# Autodesk Inventor assembly: outer
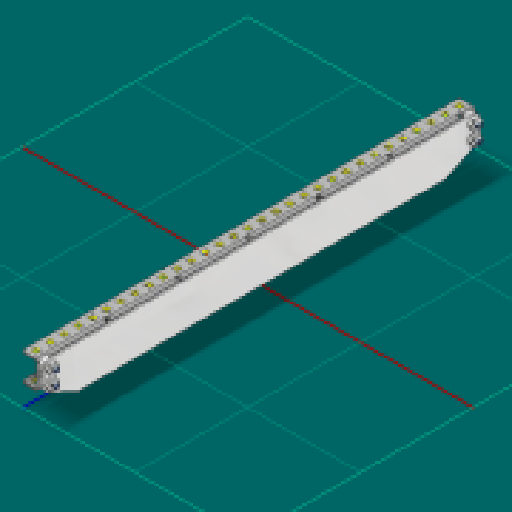
[picture p0: Inventor's stored thumbnail of the model, 512x512]
Saved by Autodesk Inventor 2025 (Build 290162000, 162)
## iProperties
Created: 2024-08-21
Part Number: outer
Document SubType Name: Assembly
Designer: averey
Author: averey
## Documents named in this file (10)
- C:\Users\avere\vex_robotics_high_stakes\hardware\cad\bots\ENIGMA\chassis\drivetrain\drivebay\outer.iam
- C:\Users\avere\vex_robotics_high_stakes\hardware\cad\VEX-CAD-Inventor\Structure\C Channel\Aluminum 1x2x1\Alu C 1x2x1x31.ipt
- C:\Users\avere\vex_robotics_high_stakes\hardware\cad\_quick_assemblies\bearing_flat_w_hardware.iam
- C:\Users\avere\vex_robotics_high_stakes\hardware\cad\bots\ENIGMA\chassis\drivetrain\drivebay\custom_parts\skirt.ipt
- C:\Users\avere\vex_robotics_high_stakes\hardware\cad\VEX-CAD-Inventor\Motion\Spacers\Spacer Nylon .500 OD\NSpacer White .500 OD x .125.ipt
- C:\Users\avere\vex_robotics_high_stakes\hardware\cad\VEX-CAD-Inventor\Motion\Spacers\Spacer Nylon .500 OD.ipt
- C:\Users\avere\vex_robotics_high_stakes\hardware\cad\VEX-CAD-Inventor\Structure\Hardware\Screw Shoulder Robosource\SScrew Shoulder Smooth .500 x .04.ipt
- C:\Users\avere\vex_robotics_high_stakes\hardware\cad\VEX-CAD-Inventor\Structure\Hardware\Screw Shoulder Robosource.ipt
- C:\Users\avere\vex_robotics_high_stakes\hardware\cad\VEX-CAD-Inventor\Structure\Hardware\Nut Nylon\Nut Nylon - White.ipt
- C:\Users\avere\vex_robotics_high_stakes\hardware\cad\VEX-CAD-Inventor\Structure\Hardware\Nut Nylon.ipt
## Components (23 placed, 6 different names)
1. Alu C 1x2x1x31:1 — Mate:1, Mate:2, Insert:1, Mate:3, Insert:3, Insert:4
2. skirt:1 — Insert:2, Insert:5
3. bearing_flat_w_hardware:1 [sub-assembly] — Insert:1, Mate:3
4. bearing_flat_w_hardware:2 [sub-assembly]
5. bearing_flat_w_hardware:3 [sub-assembly]
6. bearing_flat_w_hardware:4 [sub-assembly]
7. bearing_flat_w_hardware:5 [sub-assembly]
8. bearing_flat_w_hardware:6 [sub-assembly]
9. bearing_flat_w_hardware:7 [sub-assembly]
10. bearing_flat_w_hardware:8 [sub-assembly]
11. bearing_flat_w_hardware:9 [sub-assembly]
12. NSpacer White .500 OD x .125:1 — Insert:2, Insert:3
13. SScrew Shoulder Smooth .500 x .04:1 — Insert:4
14. Nut Nylon - White:1 — Insert:5
15. NSpacer White .500 OD x .125:2
16. SScrew Shoulder Smooth .500 x .04:2
17. Nut Nylon - White:2
18. NSpacer White .500 OD x .125:3
19. SScrew Shoulder Smooth .500 x .04:3
20. Nut Nylon - White:3
21. NSpacer White .500 OD x .125:4
22. SScrew Shoulder Smooth .500 x .04:4
23. Nut Nylon - White:4
## Component patterns: Bearings (9 elements), Hardware (4 elements)
## Relationships (8: Insert 5, Mate 3)
- Mate:1: Alu C 1x2x1x31:1
- Mate:2 (11.1125 mm): Alu C 1x2x1x31:1
- Insert:1: Alu C 1x2x1x31:1 ↔ bearing_flat_w_hardware:1
- Mate:3: Alu C 1x2x1x31:1 ↔ bearing_flat_w_hardware:1
- Insert:2: skirt:1 ↔ NSpacer White .500 OD x .125:1
- Insert:3: Alu C 1x2x1x31:1 ↔ NSpacer White .500 OD x .125:1
- Insert:4: Alu C 1x2x1x31:1 ↔ SScrew Shoulder Smooth .500 x .04:1
- Insert:5: skirt:1 ↔ Nut Nylon - White:1
